# Autodesk Inventor assembly: Assembly3
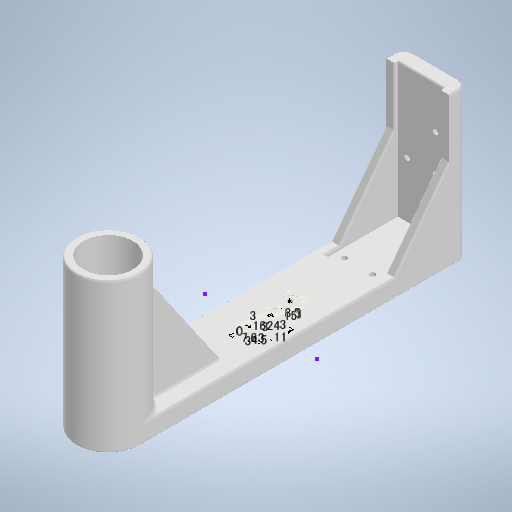
[picture p0: Inventor's stored thumbnail of the model, 512x512]
Saved by Autodesk Inventor 2025.2 (Build 292293000, 293)
## iProperties
Created: 2025-05-29
Part Number: Assembly3
Document SubType Name: Assembly
Designer: mahhy
Author: mahhy
## Documents named in this file (3)
- D:\兵庫県立大\部活\鳥人間部\Assembly3.iam
- D:\兵庫県立大\部活\鳥人間部\arm-1.ipt
- C:\Users\mahhy\Downloads\ServoMotor_Hone2 (1).ipt
## Components (2 placed, 2 different names)
1. arm-1:1 — 回転:1
2. ServoMotor_Hone2 (1):1 — 回転:1
## Relationships (1: RevoluteJoint 1)
- 回転:1 [RevoluteJoint]: arm-1:1 ↔ ServoMotor_Hone2 (1):1
